# Autodesk Inventor assembly: 12
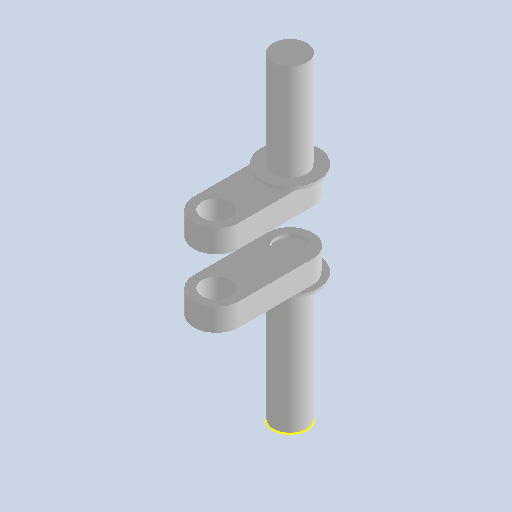
[picture p0: Inventor's stored thumbnail of the model, 512x512]
Saved by Autodesk Inventor 2025.1 (Build 291241000, 241)
## iProperties
Created: 2024-09-13
Part Number: 12
Document SubType Name: Assembly
Designer: ffogue
Author: ffogue
## Documents named in this file (5)
- C:\Users\ffogue\Documents\Inventor\Single cylinder Steam Engine\12.iam
- C:\Users\ffogue\Documents\Inventor\Single cylinder Steam Engine\12.ipt
- C:\Users\ffogue\Documents\Inventor\Single cylinder Steam Engine\sicherung.ipt
- C:\Users\ffogue\Documents\Inventor\Single cylinder Steam Engine\welle 21.ipt
- C:\Users\ffogue\Documents\Inventor\Single cylinder Steam Engine\welle 30.ipt
## Components (6 placed, 4 different names)
1. 12:1 — Mate:1, Mate:5, Insert:4, Flush:1
2. 12:2 — Mate:1, Insert:3, Flush:1
3. sicherung:1 — Mate:4, Insert:3, Mate:6, Insert:5
4. sicherung:2 — Mate:4, Mate:5, Insert:4, Mate:7, Insert:6
5. welle 21:1 — Mate:6, Insert:5
6. welle 30:1 — Mate:7, Insert:6
## Relationships (10: Mate 5, Insert 4, Flush 1)
- Mate:1: 12:1 ↔ 12:2
- Mate:4: sicherung:1 ↔ sicherung:2
- Mate:5: 12:1 ↔ sicherung:2
- Insert:3: 12:2 ↔ sicherung:1
- Insert:4: 12:1 ↔ sicherung:2
- Mate:6: sicherung:1 ↔ welle 21:1
- Insert:5: sicherung:1 ↔ welle 21:1
- Mate:7: sicherung:2 ↔ welle 30:1
- Insert:6: sicherung:2 ↔ welle 30:1
- Flush:1 (12 mm): 12:1 ↔ 12:2
